# Autodesk Inventor assembly: Bellamy_Calosc
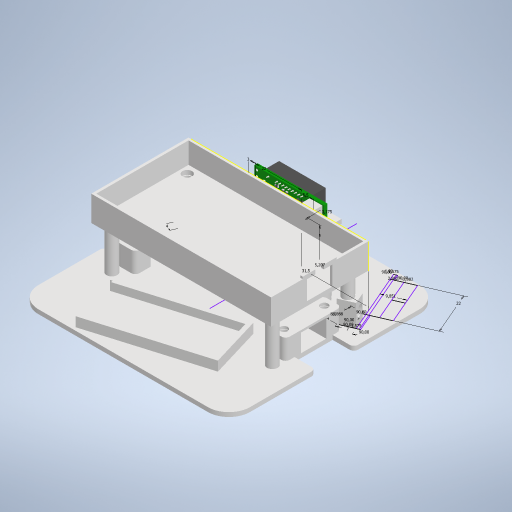
[picture p0: Inventor's stored thumbnail of the model, 512x512]
Saved by Autodesk Inventor 2023 (Build 270158000, 158)
## iProperties
Created: 2023-04-09
Part Number: Bellamy_Calosc
Document SubType Name: Assembly
Designer: julia
Author: julia
## Documents named in this file (5)
- C:\Users\julia\OneDrive\Pulpit\Inventor\Bellamy_3D-main\Do wydruku\Wydruk\Bellamy_Calosc.iam
- C:\Users\julia\OneDrive\Pulpit\Inventor\Bellamy_3D-main\cialo_nowe.ipt
- C:\Users\julia\OneDrive\Pulpit\Inventor\Bellamy_3D-main\Do wydruku\Wydruk\Pojemnik-Silnik.ipt
- C:\Users\julia\OneDrive\Pulpit\Inventor\Bellamy_3D-main\Akumulator_.ipt
- C:\Users\julia\OneDrive\Pulpit\Inventor\Bellamy_3D-main\wzrok.ipt
## Components (5 placed, 4 different names)
1. cialo_nowe:1 — Zestawiające:1, Zestawiające:2, Zestawiające:3
2. Akumulator_:1 — Zestawiające:1, Zestawiające:4
3. Pojemnik-Silnik:1 — Zestawiające:2
4. Pojemnik-Silnik:2 — Zestawiające:3
5. wzrok:1 — Zestawiające:4
## Relationships (4: Mate 4)
- Zestawiające:1 [Mate]: cialo_nowe:1 ↔ Akumulator_:1
- Zestawiające:2 [Mate]: cialo_nowe:1 ↔ Pojemnik-Silnik:1
- Zestawiające:3 [Mate]: cialo_nowe:1 ↔ Pojemnik-Silnik:2
- Zestawiające:4 [Mate]: Akumulator_:1 ↔ wzrok:1
